# Autodesk Inventor assembly: Assembly_Cube_explosion_v2
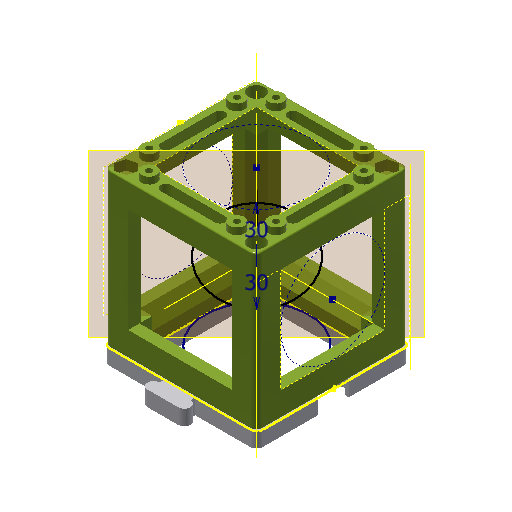
[picture p0: Inventor's stored thumbnail of the model, 512x512]
Saved by Autodesk Inventor 2022 (Build 260153000, 153)
## iProperties
Created: 2020-03-27
Part Number: Assembly_Cube_explosion_v2
Document SubType Name: Assembly
Designer: B
Mass: 27.8603 g
Surface Area: 235.464 cm^2
Volume: 27.8603 cm^3
Density: 1 g/cm^3
Author: B
## Documents named in this file (3)
- C:\Users\diederichbenedict\Dropbox\Dokumente\Promotion\PROJECTS\UC2\02_CAD\INVENTOR\uc2_v3\Assembly_Cube_empty_IM_withBase_v3.iam
- C:\Users\diederichbenedict\Dropbox\Dokumente\Promotion\PROJECTS\UC2\02_CAD\INVENTOR\uc2_v3\10_Cube_1x1_IM.ipt
- C:\Users\diederichbenedict\Dropbox\Dokumente\Promotion\PROJECTS\UC2\02_CAD\INVENTOR\uc2_v3\10_Base_puzzle_v3.ipt
## Components (3 placed, 2 different names)
1. 10_Cube_1x1_IM:1 — Mate:1, Angle:1, Mate:2, Mate:4
2. 10_Cube_1x1_IM:2 — Flush:1, Flush:2, Flush:3, Mate:1, Angle:1, Mate:2, Mate:3, Angle:2
3. 10_Base_puzzle_v3:1 — Mate:3, Mate:4, Angle:2
## Relationships (9: Mate 4, Flush 3, Angle 2)
- Flush:1: 10_Cube_1x1_IM:2
- Flush:2: 10_Cube_1x1_IM:2
- Flush:3: 10_Cube_1x1_IM:2
- Mate:1: 10_Cube_1x1_IM:1 ↔ 10_Cube_1x1_IM:2
- Angle:1 (0 deg): 10_Cube_1x1_IM:1 ↔ 10_Cube_1x1_IM:2
- Mate:2 (-50 mm): 10_Cube_1x1_IM:1 ↔ 10_Cube_1x1_IM:2
- Mate:3: 10_Cube_1x1_IM:2 ↔ 10_Base_puzzle_v3:1
- Mate:4: 10_Cube_1x1_IM:1 ↔ 10_Base_puzzle_v3:1
- Angle:2 (0 deg): 10_Cube_1x1_IM:2 ↔ 10_Base_puzzle_v3:1
